# Autodesk Inventor assembly: Knob Assembled
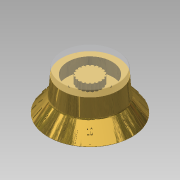
[picture p0: Inventor's stored thumbnail of the model, 180x180]
Saved by Autodesk Inventor 2016 (Build 200138000, 138)
## iProperties
Created: 2018-09-15
Part Number: Knob Assembled
Document SubType Name: Assembly
Designer: Pedro Mendonça
Author: Pedro Mendonça
## Documents named in this file (3)
- C:\Users\Pedro\Google Drive\Projeto CAD Eng Mecânica\Knob Assembled.iam
- C:\Users\Pedro\Google Drive\Projeto CAD Eng Mecânica\Knob.ipt
- C:\Users\Pedro\Google Drive\Projeto CAD Eng Mecânica\Knob (tampa).ipt
## Components (2 placed, 2 different names)
1. Knob:1 — Mate:1
2. Knob (tampa):1 — Mate:1
## Relationships (1: Mate 1)
- Mate:1: Knob:1 ↔ Knob (tampa):1
